# Autodesk Inventor assembly: Assembled
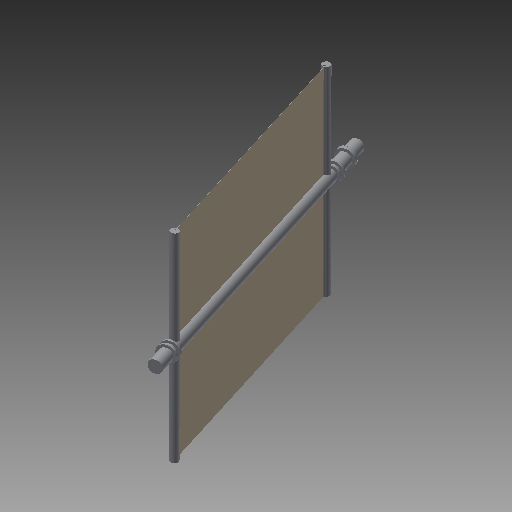
[picture p0: Inventor's stored thumbnail of the model, 512x512]
Saved by Autodesk Inventor 2018 (Build 220112000, 112)
## iProperties
Created: 2016-07-02
Part Number: Assembled
Document SubType Name: Assembly
Designer: Tore Den Store
Author: Tore Den Store
## Documents named in this file (3)
- C:\Users\ToreDenStore\Documents\Inventor\Vertical axis wind turbine\1 of 4 part\SailBeam.iam
- C:\Users\ToreDenStore\Documents\Inventor\Vertical axis wind turbine\1 of 4 part\CentralBeam.ipt
- C:\Users\ToreDenStore\Documents\Inventor\Vertical axis wind turbine\1 of 4 part\Sail.ipt
## Components (3 placed, 2 different names)
1. CentralBeam:1 — Rotational:1, Mate:1, Rotational:2, Mate:2
2. Sail:1 — Rotational:1, Mate:1
3. Sail:2 — Rotational:2, Mate:2
## Relationships (4: RevoluteJoint 2, Mate 2)
- Rotational:1 [RevoluteJoint]: CentralBeam:1 ↔ Sail:1
- Mate:1: CentralBeam:1 ↔ Sail:1
- Rotational:2 [RevoluteJoint]: CentralBeam:1 ↔ Sail:2
- Mate:2: CentralBeam:1 ↔ Sail:2
